# Autodesk Inventor assembly: BlockWedge
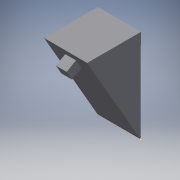
[picture p0: Inventor's stored thumbnail of the model, 180x180]
Saved by Autodesk Inventor 2016 (Build 200138000, 138)
## iProperties
Created: 2015-09-10
Part Number: BlockWedge
Document SubType Name: Assembly
Designer: Kiran
Mass: 18.3069 g
Surface Area: 53.5947 cm^2
Volume: 18.3069 cm^3
Density: 1 g/cm^3
Author: Kiran
## Documents named in this file (3)
- C:\Users\nightstalker\Downloads\ENPM 808M\WedgeBlock\BlockWedge.iam
- C:\Users\nightstalker\Downloads\ENPM 808M\WedgeBlock\Block.ipt
- C:\Users\nightstalker\Downloads\ENPM 808M\WedgeBlock\Wedge.ipt
## Components (2 placed, 2 different names)
1. Block:1 — Mate:1
2. Wedge:1 — Mate:1, Mate:2
## Relationships (2: Mate 2)
- Mate:1: Block:1 ↔ Wedge:1
- Mate:2: Wedge:1
